# Autodesk Inventor assembly: Ensamblaje2
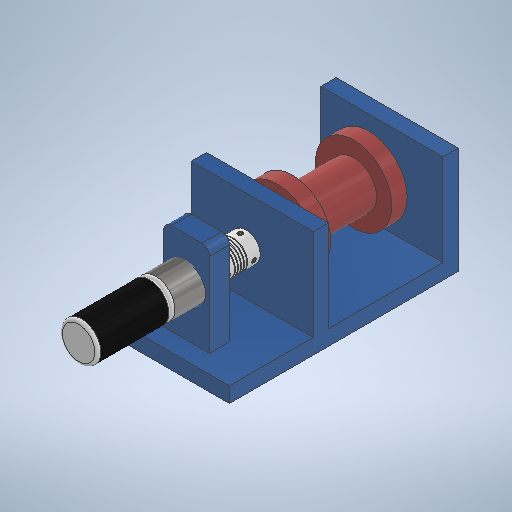
[picture p0: Inventor's stored thumbnail of the model, 512x512]
Saved by Autodesk Inventor 2026 (Build 300175050, 175E)
## iProperties
Created: 2025-06-30
Part Number: Ensamblaje2
Document SubType Name: Assembly
Designer: piero
Author: piero
## Documents named in this file (11)
- C:\Users\piero\OneDrive\Documentos\UTEC\Ciclo 2025-1\PFC_1\ModeloBase\CAD\Ensamblaje2 - V2.iam
- C:\Users\piero\OneDrive\Documentos\UTEC\Ciclo 2025-1\PFC_1\ModeloBase\acople_suave.ipt
- C:\Users\piero\OneDrive\Documentos\UTEC\Ciclo 2025-1\PFC_1\ModeloBase\Stepper Motor Nema 17_.ipt
- C:\Users\piero\OneDrive\Documentos\UTEC\Ciclo 2025-1\PFC_1\ModeloBase\Roda-608\w_608-2rs1.iam
- C:\Users\piero\OneDrive\Documentos\UTEC\Ciclo 2025-1\PFC_1\ModeloBase\Brida1.ipt
- C:\Users\piero\OneDrive\Documentos\Inventor\Content Center Files\R2026\es-ES\AS 1421(4)\AS 1421 - M3 x 4 Punta plana.ipt
- C:\Users\piero\OneDrive\Documentos\UTEC\Ciclo 2025-1\PFC_1\ModeloBase\CAD\soporte_inferior_V2.ipt
- C:\Users\piero\OneDrive\Documentos\UTEC\Ciclo 2025-1\PFC_1\ModeloBase\CAD\carrete - V2.ipt
- C:\Users\piero\OneDrive\Documentos\UTEC\Ciclo 2025-1\PFC_1\ModeloBase\CAD\perno_pasante.ipt
- C:\Users\piero\OneDrive\Documentos\UTEC\Ciclo 2025-1\PFC_1\ModeloBase\CAD\Motor.ipt
- C:\Users\piero\OneDrive\Documentos\UTEC\Ciclo 2025-1\PFC_1\ModeloBase\CAD\placa_soporte_motor.ipt
## Components (14 placed, 10 different names)
1. acople_suave:2 — Insertar:1, Insertar:2, Insertar:3, Coincidencia:16, Coincidencia:18, Coincidencia:21
2. Stepper Motor Nema 17_:2
3. w_608-2rs1:1 [sub-assembly] — De rotación:1
4. Brida1:1
5. Brida1:2
6. AS 1421 Punta plana - Métrico M3 x 4 Punta plana:1 — Insertar:1
7. AS 1421 Punta plana - Métrico M3 x 4 Punta plana:3 — Insertar:2
8. AS 1421 Punta plana - Métrico M3 x 4 Punta plana:4 — Insertar:3
9. AS 1421 Punta plana - Métrico M3 x 4 Punta plana:5 — Coincidencia:16
10. soporte_inferior_V2:1 — De rotación:1, Coincidencia:19
11. carrete - V2:1 — Coincidencia:17
12. perno_pasante:1 — Coincidencia:17, Coincidencia:18
13. Motor:1 — Coincidencia:19, Coincidencia:20, Coincidencia:21
14. placa_soporte_motor:1 — Coincidencia:20
## Relationships (10: Mate 6, Insert 3, RevoluteJoint 1)
- Insertar:1: acople_suave:2 ↔ AS 1421 Punta plana - Métrico M3 x 4 Punta plana:1
- Insertar:2: acople_suave:2 ↔ AS 1421 Punta plana - Métrico M3 x 4 Punta plana:3
- Insertar:3: acople_suave:2 ↔ AS 1421 Punta plana - Métrico M3 x 4 Punta plana:4
- Coincidencia:16 [Mate]: acople_suave:2 ↔ AS 1421 Punta plana - Métrico M3 x 4 Punta plana:5
- De rotación:1 [RevoluteJoint]: w_608-2rs1:1 ↔ soporte_inferior_V2:1
- Coincidencia:17 [Mate]: carrete - V2:1 ↔ perno_pasante:1
- Coincidencia:18 [Mate]: acople_suave:2 ↔ perno_pasante:1
- Coincidencia:19 [Mate]: soporte_inferior_V2:1 ↔ Motor:1
- Coincidencia:20 [Mate]: Motor:1 ↔ placa_soporte_motor:1
- Coincidencia:21 [Mate]: acople_suave:2 ↔ Motor:1
